# Autodesk Inventor assembly: Raspberry Pi 3
(part 2 of 2)
517. Raspberry Pi 3141_smaller_517
518. Raspberry Pi 3141_smaller_518
519. Raspberry Pi 3141_smaller_519
520. Raspberry Pi 3141_smaller_520
521. Raspberry Pi 3141_smaller_521
522. Raspberry Pi 3141_smaller_522
523. Raspberry Pi 3141_smaller_523
524. Raspberry Pi 3141_smaller_524
525. Raspberry Pi 3141_smaller_525
526. Raspberry Pi 3141_smaller_526
527. Raspberry Pi 3141_smaller_527
528. Raspberry Pi 3141_smaller_528
529. Raspberry Pi 3141_529
530. Raspberry Pi 345_530
531. Raspberry Pi 345_531
532. Raspberry Pi 345_532
533. Raspberry Pi 345_533
534. Raspberry Pi 3141_smaller_534
535. Solder2_535
536. Solder2_536
537. Solder2_537
538. Solder2_538
539. Solder2_539
540. Solder2_540
541. Solder2_541
542. Solder2_542
543. Solder2_543
544. Solder2_544
545. Solder2_545
546. Solder2_546
547. Solder2_547
548. Solder2_548
549. Solder2_549
550. Solder2_550
551. Solder2_551
552. Solder2_552
553. Solder2_553
554. Solder2_554
555. Solder2_555
556. Solder2_556
557. Solder2_557
558. Solder2_558
559. Solder2_559
560. Solder2_560
561. Solder2_561
562. Solder2_562
563. Solder2_563
564. Solder2_564
565. Solder2_565
566. Solder2_566
567. Solder2_567
568. Solder2_568
569. Solder2_569
570. Solder2_570
571. Solder2_571
572. Solder2_572
573. Solder2_573
574. Solder2_574
575. Solder2_575
576. Solder2_576
577. Solder2_577
578. Solder2_578
579. Solder2_579
580. Solder2_580
581. Solder2_581
582. Solder2_582
583. Solder2_583
584. Solder2_584
585. Solder2_585
586. Solder2_586
587. Solder2_587
588. Solder2_588
589. Solder2_589
590. Solder2_590
591. Solder2_591
592. Solder2_592
593. Solder2_593
594. raspberry_pi_B+_(microsd2)_594
595. Raspberry Pi 3242_595
596. Raspberry Pi 3242_596
597. Raspberry Pi 3242_597
598. Raspberry Pi 3242_598
599. Raspberry Pi 3242_599
600. Raspberry Pi 3242_600
601. Raspberry Pi 3242_601
602. Raspberry Pi 3242_602
603. Raspberry Pi 3242_603
604. Raspberry Pi 3242_604
605. Raspberry Pi 3242_605
606. Raspberry Pi 3242_606
607. Raspberry Pi 3242_607
608. Raspberry Pi 3242_608
609. Raspberry Pi 3242_609
610. Raspberry Pi 3242_610
611. Raspberry Pi 3242_611
612. Raspberry Pi 3242_612
613. Raspberry Pi 3242_613
614. Raspberry Pi 3266_614
615. Raspberry Pi 3266_615
616. Raspberry Pi 3266_616
617. Raspberry Pi 3266_617
618. Raspberry Pi 3266_618
619. Raspberry Pi 3266_619
620. Raspberry Pi 3266_620
621. Raspberry Pi 3266_621
622. Raspberry Pi 3266_622
623. Raspberry Pi 3266_623
624. Raspberry Pi 3266_624
625. Raspberry Pi 3266_625
626. Raspberry Pi 3266_626
627. Raspberry Pi 3266_627
628. Raspberry Pi 3266_628
629. Raspberry Pi 3266_629
630. Raspberry Pi 3266_630
631. Raspberry Pi 3266_631
632. Raspberry Pi 3266_632
633. raspberry_pi_B_(RJ45)_633
